# Autodesk Inventor assembly: GI - 100
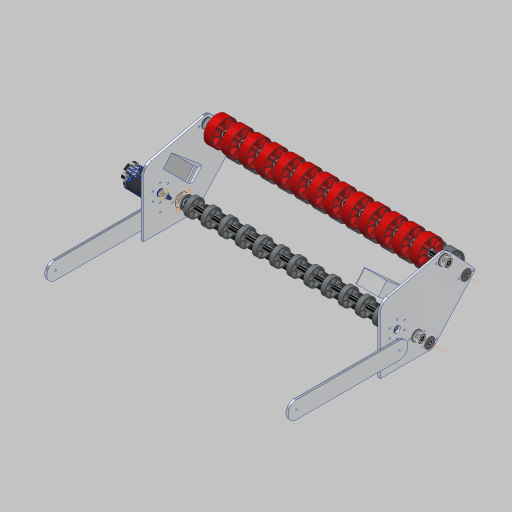
[picture p0: Inventor's stored thumbnail of the model, 512x512]
Saved by Autodesk Inventor 2023.5 (Build 275446000, 446)
## iProperties
Created: 2025-01-18
Part Number: GI - 100
Document SubType Name: Assembly
Designer: mavericks
Author: mavericks
## Documents named in this file (15)
- C:\Users\slick\OneDrive\Desktop\2025-ReefScape---CAD\ground intake\GI - 100.iam
- C:\Users\slick\OneDrive\Desktop\2025-ReefScape---CAD\ground intake\GI1\GI - 001.ipt
- C:\Users\slick\OneDrive\Desktop\2025-ReefScape---CAD\COMMON PARTS\BEARINGS\13_75mm_1_2_ThunderHex_ID_x_1_125_OD_x_0_313_WD_Flanged_Bearing_217-4006_MIR.ipt
- C:\Users\slick\OneDrive\Desktop\2025-ReefScape---CAD\ground intake\GI1\GI - 002.ipt
- C:\Users\slick\OneDrive\Desktop\2025-ReefScape---CAD\COMMON PARTS\WHEELS\am-3946 3IN 375Hex Compliant Wheel REV 3.ipt
- C:\Users\slick\OneDrive\Desktop\2025-ReefScape---CAD\COMMON PARTS\WHEELS\2_OD_Straight_Flex_Wheel_217-6354.ipt
- C:\Users\slick\OneDrive\Desktop\2025-ReefScape---CAD\ground intake\GI - 200.iam
- C:\Users\slick\OneDrive\Desktop\2025-ReefScape---CAD\COMMON PARTS\MOTORS\Kracken with Cover and Boards.iam
- C:\Users\slick\OneDrive\Desktop\2025-ReefScape---CAD\COMMON PARTS\PULLEYS\gt2\16T Gt2 Kracken PullyWCP-1178.ipt
- C:\Users\slick\OneDrive\Desktop\2025-ReefScape---CAD\COMMON PARTS\PULLEYS\gt2\24t_x_9mm_Wide_Double_Flange_Aluminum_Pulley_GT2_3mm_1_2_Hex_Bore_217-5875.ipt
- C:\Users\slick\OneDrive\Desktop\2025-ReefScape---CAD\COMMON PARTS\PULLEYS\gt2\36t_x_9mm_Wide_Double_Flange_Aluminum_Pulley_GT2_3mm_1_2_Hex_Bore_217-5873.ipt
- C:\Users\slick\OneDrive\Desktop\2025-ReefScape---CAD\ground intake\GI1\GI - 005.ipt
- C:\Users\slick\OneDrive\Desktop\2025-ReefScape---CAD\ground intake\GI1\GI - 006.ipt
- C:\Users\slick\OneDrive\Desktop\2025-ReefScape---CAD\ground intake\GI1\GI - 300.iam
- C:\Users\slick\OneDrive\Desktop\2025-ReefScape---CAD\COMMON PARTS\WHEELS\3_OD_Straight_Flex_Wheel_217-6448.ipt
## Components (66 placed, 14 different names)
1. GI - 001:1 — Insert:1, Insert:2, Insert:3, Insert:4, Mate:4, Mate:6, Insert:18, Mate:7, Mate:15, Mate:28, Angle:1, Insert:21, Mate:35
2. 13_75mm_1_2_ThunderHex_ID_x_1_125_OD_x_0_313_WD_Flanged_Bearing_217-4006_MIR:1 — Insert:2, Mate:15, Mate:25, Mate:26
3. 13_75mm_1_2_ThunderHex_ID_x_1_125_OD_x_0_313_WD_Flanged_Bearing_217-4006_MIR:2 — Insert:1, Mate:3, Flush:4, Mate:23, Mate:24
4. 13_75mm_1_2_ThunderHex_ID_x_1_125_OD_x_0_313_WD_Flanged_Bearing_217-4006_MIR:3 — Insert:4, Insert:19
5. 13_75mm_1_2_ThunderHex_ID_x_1_125_OD_x_0_313_WD_Flanged_Bearing_217-4006_MIR:4 — Insert:3, Mate:5, Mate:10, Mate:11, Mate:12, Mate:20, Mate:21
6. GI - 001:2 — Insert:5, Insert:6, Insert:7, Insert:8, Mate:29, Insert:20, Angle:2
7. 13_75mm_1_2_ThunderHex_ID_x_1_125_OD_x_0_313_WD_Flanged_Bearing_217-4006_MIR:5 — Insert:5, Mate:33, Flush:9
8. 13_75mm_1_2_ThunderHex_ID_x_1_125_OD_x_0_313_WD_Flanged_Bearing_217-4006_MIR:6 — Insert:6, Mate:18
9. 13_75mm_1_2_ThunderHex_ID_x_1_125_OD_x_0_313_WD_Flanged_Bearing_217-4006_MIR:7 — Insert:8, Insert:16, Mate:14
10. 13_75mm_1_2_ThunderHex_ID_x_1_125_OD_x_0_313_WD_Flanged_Bearing_217-4006_MIR:8 — Insert:7
11. GI - 002:1 — Mate:18, Flush:4, Mate:27
12. GI - 002:2 — Mate:17, Flush:3, Mate:20, Mate:21
13. GI - 200:1 [sub-assembly] — Insert:16, Mate:13, Insert:19
14. Kracken with Cover and Boards:1 [sub-assembly] — Insert:18, Mate:7, Mate:8, Mate:9, Mate:32
15. 16T Gt2 Kracken PullyWCP-1178:1 — Mate:8, Mate:9
16. 24t_x_9mm_Wide_Double_Flange_Aluminum_Pulley_GT2_3mm_1_2_Hex_Bore_217-5875:1 — Mate:10, Flush:1
17. 36t_x_9mm_Wide_Double_Flange_Aluminum_Pulley_GT2_3mm_1_2_Hex_Bore_217-5873:1 — Mate:11, Mate:12
18. 24t_x_9mm_Wide_Double_Flange_Aluminum_Pulley_GT2_3mm_1_2_Hex_Bore_217-5875:2 — Mate:13, Mate:14, Flush:1
19. 24t_x_9mm_Wide_Double_Flange_Aluminum_Pulley_GT2_3mm_1_2_Hex_Bore_217-5875:3 — Mate:17, Flush:3
20. 24t_x_9mm_Wide_Double_Flange_Aluminum_Pulley_GT2_3mm_1_2_Hex_Bore_217-5875:4 — Mate:27
21. 24t_x_9mm_Wide_Double_Flange_Aluminum_Pulley_GT2_3mm_1_2_Hex_Bore_217-5875:5 — Mate:23, Mate:24
22. 24t_x_9mm_Wide_Double_Flange_Aluminum_Pulley_GT2_3mm_1_2_Hex_Bore_217-5875:6 — Mate:25, Mate:26
23. GI - 005:1 — Mate:28, Flush:7, Angle:1, Mate:32
24. GI - 005:2 — Mate:29, Flush:7
25. GI - 006:1 — Insert:20, Angle:2, Flush:8
26. GI - 006:2 — Insert:21, Flush:8
27. GI - 300:1 [sub-assembly] — Mate:33, Flush:9, Mate:34
28. am-3946 3IN 375Hex Compliant Wheel REV 3:1 — Mate:3, Mate:4
29. am-3946 3IN 375Hex Compliant Wheel REV 3:2
30. am-3946 3IN 375Hex Compliant Wheel REV 3:3
31. am-3946 3IN 375Hex Compliant Wheel REV 3:4
32. am-3946 3IN 375Hex Compliant Wheel REV 3:5
33. am-3946 3IN 375Hex Compliant Wheel REV 3:6
34. am-3946 3IN 375Hex Compliant Wheel REV 3:7
35. am-3946 3IN 375Hex Compliant Wheel REV 3:8
36. am-3946 3IN 375Hex Compliant Wheel REV 3:9
37. am-3946 3IN 375Hex Compliant Wheel REV 3:10
38. am-3946 3IN 375Hex Compliant Wheel REV 3:11
39. am-3946 3IN 375Hex Compliant Wheel REV 3:12
40. am-3946 3IN 375Hex Compliant Wheel REV 3:13
41. 2_OD_Straight_Flex_Wheel_217-6354:1 — Mate:5, Mate:6
42. 2_OD_Straight_Flex_Wheel_217-6354:2
43. 2_OD_Straight_Flex_Wheel_217-6354:3
44. 2_OD_Straight_Flex_Wheel_217-6354:4
45. 2_OD_Straight_Flex_Wheel_217-6354:5
46. 2_OD_Straight_Flex_Wheel_217-6354:6
47. 2_OD_Straight_Flex_Wheel_217-6354:7
48. 2_OD_Straight_Flex_Wheel_217-6354:8
49. 2_OD_Straight_Flex_Wheel_217-6354:9
50. 2_OD_Straight_Flex_Wheel_217-6354:10
51. 2_OD_Straight_Flex_Wheel_217-6354:11
52. 2_OD_Straight_Flex_Wheel_217-6354:12
53. 2_OD_Straight_Flex_Wheel_217-6354:13
54. 3_OD_Straight_Flex_Wheel_217-6448:1 — Mate:34, Mate:35
55. 3_OD_Straight_Flex_Wheel_217-6448:2
56. 3_OD_Straight_Flex_Wheel_217-6448:3
57. 3_OD_Straight_Flex_Wheel_217-6448:4
58. 3_OD_Straight_Flex_Wheel_217-6448:5
59. 3_OD_Straight_Flex_Wheel_217-6448:6
60. 3_OD_Straight_Flex_Wheel_217-6448:7
61. 3_OD_Straight_Flex_Wheel_217-6448:8
62. 3_OD_Straight_Flex_Wheel_217-6448:9
63. 3_OD_Straight_Flex_Wheel_217-6448:10
64. 3_OD_Straight_Flex_Wheel_217-6448:11
65. 3_OD_Straight_Flex_Wheel_217-6448:12
66. 3_OD_Straight_Flex_Wheel_217-6448:13
## Component patterns: (13 elements, first: am-3946 3IN 375Hex Compliant Wheel REV 3:1), (13 elements, first: 2_OD_Straight_Flex_Wheel_217-6354:1), (13 elements, first: 3_OD_Straight_Flex_Wheel_217-6448:1)
## Relationships (49: Mate 28, Insert 13, Flush 6, Angle 2)
- Insert:1: GI - 001:1 ↔ 13_75mm_1_2_ThunderHex_ID_x_1_125_OD_x_0_313_WD_Flanged_Bearing_217-4006_MIR:2
- Insert:2: GI - 001:1 ↔ 13_75mm_1_2_ThunderHex_ID_x_1_125_OD_x_0_313_WD_Flanged_Bearing_217-4006_MIR:1
- Insert:3: GI - 001:1 ↔ 13_75mm_1_2_ThunderHex_ID_x_1_125_OD_x_0_313_WD_Flanged_Bearing_217-4006_MIR:4
- Insert:4: GI - 001:1 ↔ 13_75mm_1_2_ThunderHex_ID_x_1_125_OD_x_0_313_WD_Flanged_Bearing_217-4006_MIR:3
- Insert:5: GI - 001:2 ↔ 13_75mm_1_2_ThunderHex_ID_x_1_125_OD_x_0_313_WD_Flanged_Bearing_217-4006_MIR:5
- Insert:6: GI - 001:2 ↔ 13_75mm_1_2_ThunderHex_ID_x_1_125_OD_x_0_313_WD_Flanged_Bearing_217-4006_MIR:6
- Insert:7: GI - 001:2 ↔ 13_75mm_1_2_ThunderHex_ID_x_1_125_OD_x_0_313_WD_Flanged_Bearing_217-4006_MIR:8
- Insert:8: GI - 001:2 ↔ 13_75mm_1_2_ThunderHex_ID_x_1_125_OD_x_0_313_WD_Flanged_Bearing_217-4006_MIR:7
- Mate:3: 13_75mm_1_2_ThunderHex_ID_x_1_125_OD_x_0_313_WD_Flanged_Bearing_217-4006_MIR:2 ↔ am-3946 3IN 375Hex Compliant Wheel REV 3:1
- Mate:4 (30.1625 mm): GI - 001:1 ↔ am-3946 3IN 375Hex Compliant Wheel REV 3:1
- Mate:5: 13_75mm_1_2_ThunderHex_ID_x_1_125_OD_x_0_313_WD_Flanged_Bearing_217-4006_MIR:4 ↔ 2_OD_Straight_Flex_Wheel_217-6354:1
- Mate:6 (36.5125 mm): GI - 001:1 ↔ 2_OD_Straight_Flex_Wheel_217-6354:1
- Insert:16: 13_75mm_1_2_ThunderHex_ID_x_1_125_OD_x_0_313_WD_Flanged_Bearing_217-4006_MIR:7 ↔ GI - 200:1
- Insert:18: GI - 001:1 ↔ Kracken with Cover and Boards:1
- Mate:7: GI - 001:1 ↔ Kracken with Cover and Boards:1
- Mate:8: Kracken with Cover and Boards:1 ↔ 16T Gt2 Kracken PullyWCP-1178:1
- Mate:9 (3.175 mm): Kracken with Cover and Boards:1 ↔ 16T Gt2 Kracken PullyWCP-1178:1
- Mate:10: 13_75mm_1_2_ThunderHex_ID_x_1_125_OD_x_0_313_WD_Flanged_Bearing_217-4006_MIR:4 ↔ 24t_x_9mm_Wide_Double_Flange_Aluminum_Pulley_GT2_3mm_1_2_Hex_Bore_217-5875:1
- Mate:11: 13_75mm_1_2_ThunderHex_ID_x_1_125_OD_x_0_313_WD_Flanged_Bearing_217-4006_MIR:4 ↔ 36t_x_9mm_Wide_Double_Flange_Aluminum_Pulley_GT2_3mm_1_2_Hex_Bore_217-5873:1
- Mate:12 (3.175 mm): 13_75mm_1_2_ThunderHex_ID_x_1_125_OD_x_0_313_WD_Flanged_Bearing_217-4006_MIR:4 ↔ 36t_x_9mm_Wide_Double_Flange_Aluminum_Pulley_GT2_3mm_1_2_Hex_Bore_217-5873:1
- Mate:13: GI - 200:1 ↔ 24t_x_9mm_Wide_Double_Flange_Aluminum_Pulley_GT2_3mm_1_2_Hex_Bore_217-5875:2
- Mate:14: 13_75mm_1_2_ThunderHex_ID_x_1_125_OD_x_0_313_WD_Flanged_Bearing_217-4006_MIR:7 ↔ 24t_x_9mm_Wide_Double_Flange_Aluminum_Pulley_GT2_3mm_1_2_Hex_Bore_217-5875:2
- Flush:1: 24t_x_9mm_Wide_Double_Flange_Aluminum_Pulley_GT2_3mm_1_2_Hex_Bore_217-5875:1 ↔ 24t_x_9mm_Wide_Double_Flange_Aluminum_Pulley_GT2_3mm_1_2_Hex_Bore_217-5875:2
- Mate:15: GI - 001:1 ↔ 13_75mm_1_2_ThunderHex_ID_x_1_125_OD_x_0_313_WD_Flanged_Bearing_217-4006_MIR:1
- Insert:19: 13_75mm_1_2_ThunderHex_ID_x_1_125_OD_x_0_313_WD_Flanged_Bearing_217-4006_MIR:3 ↔ GI - 200:1
- Mate:17: GI - 002:2 ↔ 24t_x_9mm_Wide_Double_Flange_Aluminum_Pulley_GT2_3mm_1_2_Hex_Bore_217-5875:3
- Flush:3: GI - 002:2 ↔ 24t_x_9mm_Wide_Double_Flange_Aluminum_Pulley_GT2_3mm_1_2_Hex_Bore_217-5875:3
- Mate:18: 13_75mm_1_2_ThunderHex_ID_x_1_125_OD_x_0_313_WD_Flanged_Bearing_217-4006_MIR:6 ↔ GI - 002:1
- Flush:4: 13_75mm_1_2_ThunderHex_ID_x_1_125_OD_x_0_313_WD_Flanged_Bearing_217-4006_MIR:2 ↔ GI - 002:1
- Mate:20: 13_75mm_1_2_ThunderHex_ID_x_1_125_OD_x_0_313_WD_Flanged_Bearing_217-4006_MIR:4 ↔ GI - 002:2
- Mate:21: 13_75mm_1_2_ThunderHex_ID_x_1_125_OD_x_0_313_WD_Flanged_Bearing_217-4006_MIR:4 ↔ GI - 002:2
- Mate:23: 13_75mm_1_2_ThunderHex_ID_x_1_125_OD_x_0_313_WD_Flanged_Bearing_217-4006_MIR:2 ↔ 24t_x_9mm_Wide_Double_Flange_Aluminum_Pulley_GT2_3mm_1_2_Hex_Bore_217-5875:5
- Mate:24 (3.175 mm): 13_75mm_1_2_ThunderHex_ID_x_1_125_OD_x_0_313_WD_Flanged_Bearing_217-4006_MIR:2 ↔ 24t_x_9mm_Wide_Double_Flange_Aluminum_Pulley_GT2_3mm_1_2_Hex_Bore_217-5875:5
- Mate:25: 13_75mm_1_2_ThunderHex_ID_x_1_125_OD_x_0_313_WD_Flanged_Bearing_217-4006_MIR:1 ↔ 24t_x_9mm_Wide_Double_Flange_Aluminum_Pulley_GT2_3mm_1_2_Hex_Bore_217-5875:6
- Mate:26 (3.175 mm): 13_75mm_1_2_ThunderHex_ID_x_1_125_OD_x_0_313_WD_Flanged_Bearing_217-4006_MIR:1 ↔ 24t_x_9mm_Wide_Double_Flange_Aluminum_Pulley_GT2_3mm_1_2_Hex_Bore_217-5875:6
- Mate:27: GI - 002:1 ↔ 24t_x_9mm_Wide_Double_Flange_Aluminum_Pulley_GT2_3mm_1_2_Hex_Bore_217-5875:4
- Mate:28: GI - 001:1 ↔ GI - 005:1
- Mate:29: GI - 001:2 ↔ GI - 005:2
- Flush:7: GI - 005:1 ↔ GI - 005:2
- Angle:1 (40 deg): GI - 001:1 ↔ GI - 005:1
- Mate:32 (57.15 mm): Kracken with Cover and Boards:1 ↔ GI - 005:1
- Insert:20: GI - 001:2 ↔ GI - 006:1
- Insert:21: GI - 001:1 ↔ GI - 006:2
- Angle:2 (0 deg): GI - 001:2 ↔ GI - 006:1
- Flush:8: GI - 006:1 ↔ GI - 006:2
- Mate:33: 13_75mm_1_2_ThunderHex_ID_x_1_125_OD_x_0_313_WD_Flanged_Bearing_217-4006_MIR:5 ↔ GI - 300:1
- Flush:9: 13_75mm_1_2_ThunderHex_ID_x_1_125_OD_x_0_313_WD_Flanged_Bearing_217-4006_MIR:5 ↔ GI - 300:1
- Mate:34: GI - 300:1 ↔ 3_OD_Straight_Flex_Wheel_217-6448:1
- Mate:35 (25.4 mm): GI - 001:1 ↔ 3_OD_Straight_Flex_Wheel_217-6448:1
